# Autodesk Inventor assembly: Screw and nut
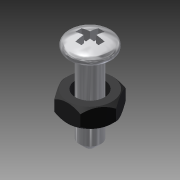
[picture p0: Inventor's stored thumbnail of the model, 180x180]
Saved by Autodesk Inventor 2015 (Build 190159000, 159)
## iProperties
Created: 2014-10-10
Part Number: Screw and nut
Document SubType Name: Assembly
Designer: lethcoec
Author: lethcoec
## Documents named in this file (3)
- \\st-svr\studenthdrives$\18\LethcoeC\IED - Lethcoe\FTC Inventor\FTC Parts\Subassemblies\Screw and nut.iam
- \\st-svr\studenthdrives$\18\LethcoeC\IED - Lethcoe\FTC Inventor\Imported Components\Screw5\Screw5.ipt
- \\st-svr\studenthdrives$\18\LethcoeC\IED - Lethcoe\FTC Inventor\Imported Components\Nut\Nut.ipt
## Components (2 placed, 2 different names)
1. Screw5:1 — Mate:1, Mate:2
2. Nut:1 — Mate:1, Mate:2
## Relationships (2: Mate 2)
- Mate:1: Screw5:1 ↔ Nut:1
- Mate:2 (4 mm): Screw5:1 ↔ Nut:1
